# Autodesk Inventor assembly: Fixture-Assembly
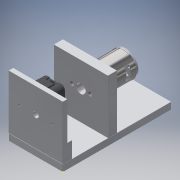
[picture p0: Inventor's stored thumbnail of the model, 180x180]
Saved by Autodesk Inventor 2016 (Build 200138000, 138)
## iProperties
Created: 2015-04-16
Part Number: Fixture-Assembly
Document SubType Name: Assembly
Designer: jonathan
Mass: 248.559 g
Surface Area: 904.248 cm^2
Volume: 248.559 cm^3
Density: 1 g/cm^3
Author: jonathan
## Documents named in this file (4)
- C:\Users\jonathan\Desktop\CLEAN COPIES\DC Motor Test Stand\Inventor\Fixture Assembly.iam
- C:\Users\jonathan\Desktop\CLEAN COPIES\DC Motor Test Stand\Inventor\Motor Fixture.iam
- C:\Users\jonathan\Desktop\CLEAN COPIES\DC Motor Test Stand\Inventor\Fixture Encoder.ipt
- C:\Users\jonathan\Desktop\CLEAN COPIES\DC Motor Test Stand\Inventor\Motor Assembly.iam
## Components (3 placed, 3 different names)
1. Motor Fixture:1 [sub-assembly] — Mate:1, Mate:2, Mate:3, Mate:4, Mate:5
2. Fixture Encoder:1 — Mate:1, Mate:2, Mate:3
3. Motor Assembly:1 [sub-assembly] — Mate:4, Mate:5
## Relationships (5: Mate 5)
- Mate:1: Motor Fixture:1 ↔ Fixture Encoder:1
- Mate:2: Motor Fixture:1 ↔ Fixture Encoder:1
- Mate:3: Motor Fixture:1 ↔ Fixture Encoder:1
- Mate:4: Motor Fixture:1 ↔ Motor Assembly:1
- Mate:5: Motor Fixture:1 ↔ Motor Assembly:1
